# Autodesk Inventor assembly: DribblerUnit
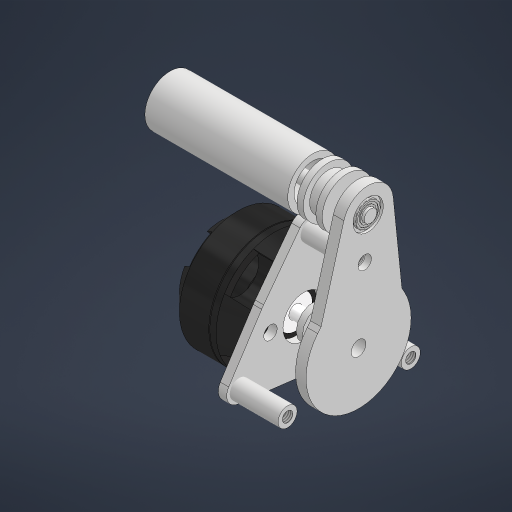
[picture p0: Inventor's stored thumbnail of the model, 512x512]
Saved by Autodesk Inventor 2024.2 (Build 282272000, 272)
## iProperties
Created: 2023-12-27
Part Number: DribblerUnit
Document SubType Name: Assembly
Designer: Hanaoka
Author: Hanaoka
## Documents named in this file (10)
- G:\共有ドライブ\reRo\05_個人\hanaoka\inventor\DribblerUnit\DribblerUnit.iam
- G:\共有ドライブ\reRo\05_個人\hanaoka\inventor\DribblerUnit\C2822_BLDC.ipt
- G:\共有ドライブ\reRo\05_個人\hanaoka\inventor\DribblerUnit\Shaft_D3.ipt
- G:\共有ドライブ\reRo\05_個人\hanaoka\inventor\DribblerUnit\tube.ipt
- G:\共有ドライブ\reRo\05_個人\hanaoka\inventor\DribblerUnit\Bearing_C-FL673ZZ.ipt
- G:\共有ドライブ\reRo\05_個人\hanaoka\inventor\DribblerUnit\Main_Frame.ipt
- G:\共有ドライブ\reRo\05_個人\hanaoka\inventor\DribblerUnit\Pulley_D3_P6.ipt
- G:\共有ドライブ\reRo\05_個人\hanaoka\inventor\DribblerUnit\Pulley_D3_P10.ipt
- G:\共有ドライブ\reRo\05_個人\hanaoka\inventor\DribblerUnit\BLDC_mount.ipt
- G:\共有ドライブ\reRo\05_個人\hanaoka\inventor\DribblerUnit\Shaf.ipt
## Components (11 placed, 9 different names)
1. C2822_BLDC:1 — 挿入:4, 挿入:6, 挿入:7, メイト:10
2. Main_Frame:1 — メイト:2, 正接:1, 挿入:4, メイト:4, メイト:5, メイト:6, メイト:12, メイト:13
3. BLDC_mount:1 — 挿入:6, 挿入:7, メイト:4, メイト:11
4. Pulley_D3_P10:1 — メイト:8
5. tube:1 — メイト:9
6. Shaft_D3:1 — メイト:7, メイト:8, メイト:9
7. Bearing_C-FL673ZZ:1 — メイト:5, メイト:6, メイト:7
8. Pulley_D3_P6:1 — メイト:10
9. Shaf:1 — メイト:11, メイト:12, メイト:13
10. Shaf:2
11. Shaf:3
## Component patterns: (3 elements, first: Shaf:1)
## Relationships (15: Mate 11, Insert 3, Tangent 1)
- メイト:2 [Mate]: Main_Frame:1
- 正接:1 [Tangent]: Main_Frame:1
- 挿入:4 [Insert]: C2822_BLDC:1 ↔ Main_Frame:1
- 挿入:6 [Insert]: C2822_BLDC:1 ↔ BLDC_mount:1
- 挿入:7 [Insert]: C2822_BLDC:1 ↔ BLDC_mount:1
- メイト:4 [Mate]: Main_Frame:1 ↔ BLDC_mount:1
- メイト:5 [Mate]: Main_Frame:1 ↔ Bearing_C-FL673ZZ:1
- メイト:6 [Mate]: Main_Frame:1 ↔ Bearing_C-FL673ZZ:1
- メイト:7 [Mate]: Shaft_D3:1 ↔ Bearing_C-FL673ZZ:1
- メイト:8 [Mate]: Pulley_D3_P10:1 ↔ Shaft_D3:1
- メイト:9 [Mate]: tube:1 ↔ Shaft_D3:1
- メイト:10 [Mate]: C2822_BLDC:1 ↔ Pulley_D3_P6:1
- メイト:11 [Mate]: BLDC_mount:1 ↔ Shaf:1
- メイト:12 [Mate]: Main_Frame:1 ↔ Shaf:1
- メイト:13 [Mate]: Main_Frame:1 ↔ Shaf:1
